# Autodesk Inventor assembly: Top
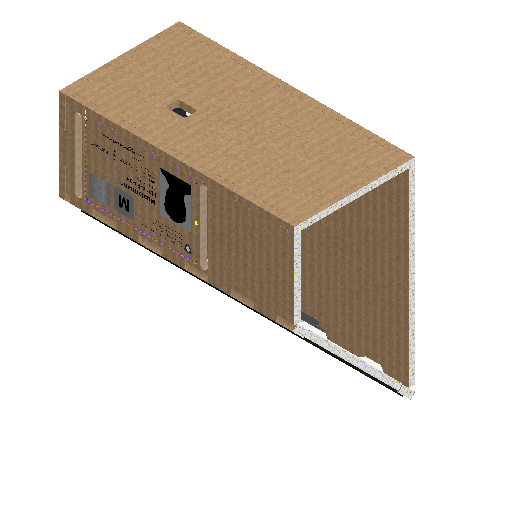
[picture p0: Inventor's stored thumbnail of the model, 512x512]
Saved by Autodesk Inventor 2025.2 (Build 292293000, 293)
## iProperties
Created: 2025-03-07
Part Number: Top
Document SubType Name: Assembly
Designer: ahorat
Author: ahorat
## Documents named in this file (11)
- C:\Daten\Temp\R32EntrySystem\cad\Top.iam
- C:\Daten\Temp\R32EntrySystem\cad\Housing\Frontplate.ipt
- C:\Daten\Temp\R32EntrySystem\cad\Housing\SidePlate.ipt
- C:\Daten\Temp\R32EntrySystem\cad\Housing\Topplate.ipt
- C:\Daten\Temp\R32EntrySystem\cad\Housing\FloorPlate.ipt
- C:\Daten\Temp\R32EntrySystem\cad\RpiTower.iam
- C:\Daten\Temp\R32EntrySystem\cad\Housing\Backplate.ipt
- C:\Daten\Temp\R32EntrySystem\cad\Rpi\raspberry pi display.iam
- C:\Daten\Temp\R32EntrySystem\cad\Housing\LED_Cover.ipt
- C:\Daten\Temp\R32EntrySystem\cad\Display_Holder.ipt
- C:\Daten\Temp\R32EntrySystem\cad\Housing\Distance_plate.ipt
## Components (12 placed, 10 different names)
1. Frontplate:1 — Flush:4, Flush:5, Mate:1, Flush:13, Mate:2, Mate:6
2. Topplate:1 — Flush:1, Flush:2, Flush:3, Flush:17, Flush:22, Flush:23, Mate:7, Mate:8, Mate:9, Mate:10
3. SidePlate:1 — Flush:1, Flush:2, Flush:3, Flush:4, Flush:10, Flush:11, Flush:12, Flush:16, Mate:6
4. FloorPlate:1 — Flush:6, Flush:7, Flush:8, Flush:10, Flush:11, Flush:12, Flush:18, Mate:4, Mate:5, Flush:21, Mate:15, Mate:16
5. raspberry pi display:2 [sub-assembly] — Mate:1, Flush:13, Mate:2, Mate:11, Mate:12, Mate:13
6. RpiTower:1 [sub-assembly] — Mate:4, Mate:5, Mate:14, Mate:17
7. Backplate:1 — Flush:16, Flush:17, Flush:18, Flush:19, Flush:20
8. SidePlate:2 — Flush:19, Flush:20, Flush:21, Flush:5
9. LED_Cover:1 — Flush:23, Mate:8, Mate:9
10. LED_Cover:2 — Flush:22, Mate:7, Mate:10
11. Display_Holder:1 — Mate:11, Mate:12, Mate:13
12. Distance_plate:1 — Mate:14, Mate:15, Mate:16, Mate:17
## Relationships (36: Flush 20, Mate 16)
- Flush:1: Topplate:1 ↔ SidePlate:1
- Flush:2: Topplate:1 ↔ SidePlate:1
- Flush:3: Topplate:1 ↔ SidePlate:1
- Flush:4: Frontplate:1 ↔ SidePlate:1
- Flush:5: Frontplate:1 ↔ SidePlate:2
- Flush:6: FloorPlate:1
- Flush:7: FloorPlate:1
- Flush:8: FloorPlate:1
- Flush:10: SidePlate:1 ↔ FloorPlate:1
- Flush:11: SidePlate:1 ↔ FloorPlate:1
- Flush:12: SidePlate:1 ↔ FloorPlate:1
- Mate:1: Frontplate:1 ↔ raspberry pi display:2
- Flush:13 (-3 mm): Frontplate:1 ↔ raspberry pi display:2
- Mate:2: Frontplate:1 ↔ raspberry pi display:2
- Flush:16: SidePlate:1 ↔ Backplate:1
- Flush:17: Topplate:1 ↔ Backplate:1
- Flush:18: FloorPlate:1 ↔ Backplate:1
- Mate:4: FloorPlate:1 ↔ RpiTower:1
- Mate:5: FloorPlate:1 ↔ RpiTower:1
- Mate:6 (0.13 mm): Frontplate:1 ↔ SidePlate:1
- Flush:19: Backplate:1 ↔ SidePlate:2
- Flush:20: Backplate:1 ↔ SidePlate:2
- Flush:21: FloorPlate:1 ↔ SidePlate:2
- Flush:22: Topplate:1 ↔ LED_Cover:2
- Flush:23: Topplate:1 ↔ LED_Cover:1
- Mate:7: Topplate:1 ↔ LED_Cover:2
- Mate:8: Topplate:1 ↔ LED_Cover:1
- Mate:9: Topplate:1 ↔ LED_Cover:1
- Mate:10: Topplate:1 ↔ LED_Cover:2
- Mate:11: raspberry pi display:2 ↔ Display_Holder:1
- Mate:12: raspberry pi display:2 ↔ Display_Holder:1
- Mate:13: raspberry pi display:2 ↔ Display_Holder:1
- Mate:14: RpiTower:1 ↔ Distance_plate:1
- Mate:15: FloorPlate:1 ↔ Distance_plate:1
- Mate:16: FloorPlate:1 ↔ Distance_plate:1
- Mate:17: RpiTower:1 ↔ Distance_plate:1
